# Autodesk Inventor assembly: 000-A-000
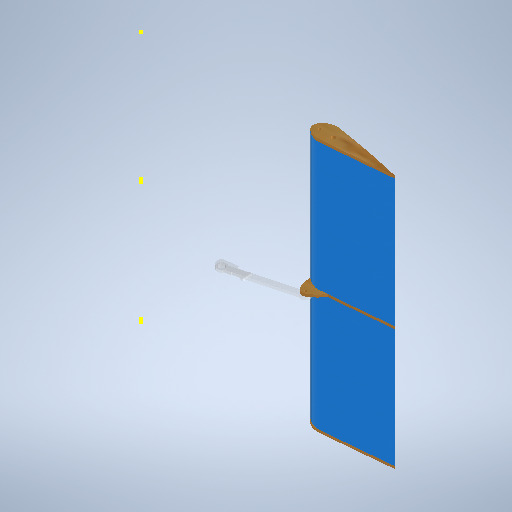
[picture p0: Inventor's stored thumbnail of the model, 512x512]
Saved by Autodesk Inventor 2025.2 (Build 292293000, 293)
## iProperties
Category: <PROJECT CATAGORY>
Created: 2025-01-30
Part Number: 000-A-000
Document SubType Name: Assembly
Designer: Carriett 4
Title: <TITLE>
Author: Carriett 4
Revision Number: A
## Documents named in this file (8)
- C:\Users\Carriett 4\OneDrive\CAD library\AILERON ASSEMBLY\FinalAssemblyAileron290125\4A.01.02.06-BC-v1-Final Aileron Assembly 80deg.iam
- C:\Users\Carriett 4\OneDrive\CAD library\AILERON ASSEMBLY\FinalAssemblyAileron290125\4P.01.02.17-BC-v1-End Ribs.ipt
- C:\Users\Carriett 4\OneDrive\CAD library\AILERON ASSEMBLY\FinalAssemblyAileron290125\4P.01.02.20-BC-v1-Middle Connecting Rib.ipt
- C:\Users\Carriett 4\OneDrive\CAD library\AILERON ASSEMBLY\FinalAssemblyAileron290125\4P.01.02.21-BC-v1-Inboard Foam Rib.ipt
- C:\Users\Carriett 4\OneDrive\CAD library\AILERON ASSEMBLY\FinalAssemblyAileron290125\4P.01.02.22-BC-v1-Outboard Foam Rib.ipt
- C:\Users\Carriett 4\OneDrive\CAD library\AILERON ASSEMBLY\FinalAssemblyAileron290125\4P.01.02.27-BC-v1-Final Aileron L2 80deg.ipt
- C:\Users\Carriett 4\OneDrive\CAD library\AILERON ASSEMBLY\FinalAssemblyAileron290125\4P.01.02.28-BC-v1-Final Aileron L3 80deg.ipt
- C:\Users\me19654\OneDrive - University of Bristol\PhD Project\005 Design (CAD and schematics)\001 Wind Tunnel\CAD Library\001-A-017 CONTRACTION ASSY.iam
## Components (7 placed, 6 different names)
1. 4P.01.02.17-BC-v1-End Ribs:1 — Rigid:4
2. 4P.01.02.17-BC-v1-End Ribs:2 — Rigid:1
3. 4P.01.02.20-BC-v1-Middle Connecting Rib:1 — Rigid:2, Rigid:3, Rotational:1
4. 4P.01.02.21-BC-v1-Inboard Foam Rib:1 — Rigid:1, Rigid:2
5. 4P.01.02.22-BC-v1-Outboard Foam Rib:1 — Rigid:3, Rigid:4
6. 4P.01.02.27-BC-v1-Final Aileron L2 80deg:1 — Rotational:2
7. 4P.01.02.28-BC-v1-Final Aileron L3 80deg:1 — Rotational:1, Rotational:2
## Relationships (6: WeldJoint 4, RevoluteJoint 2)
- Rigid:1 [WeldJoint]: 4P.01.02.17-BC-v1-End Ribs:2 ↔ 4P.01.02.21-BC-v1-Inboard Foam Rib:1
- Rigid:2 [WeldJoint]: 4P.01.02.20-BC-v1-Middle Connecting Rib:1 ↔ 4P.01.02.21-BC-v1-Inboard Foam Rib:1
- Rigid:3 [WeldJoint]: 4P.01.02.20-BC-v1-Middle Connecting Rib:1 ↔ 4P.01.02.22-BC-v1-Outboard Foam Rib:1
- Rigid:4 [WeldJoint]: 4P.01.02.17-BC-v1-End Ribs:1 ↔ 4P.01.02.22-BC-v1-Outboard Foam Rib:1
- Rotational:1 [RevoluteJoint]: 4P.01.02.20-BC-v1-Middle Connecting Rib:1 ↔ 4P.01.02.28-BC-v1-Final Aileron L3 80deg:1
- Rotational:2 [RevoluteJoint]: 4P.01.02.27-BC-v1-Final Aileron L2 80deg:1 ↔ 4P.01.02.28-BC-v1-Final Aileron L3 80deg:1
